# Autodesk Inventor assembly: servoMount
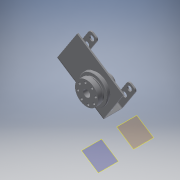
[picture p0: Inventor's stored thumbnail of the model, 180x180]
Saved by Autodesk Inventor 2017 (Build 210142000, 142)
## iProperties
Created: 2017-03-22
Part Number: servoMount
Document SubType Name: Assembly
Designer: admin
Author: admin
## Documents named in this file (5)
- C:\Users\admin\Desktop\CAD\servoMount.iam
- C:\Users\admin\Downloads\bearing.ipt
- C:\Users\admin\Downloads\hub.ipt
- C:\Users\admin\Downloads\Hitec HS-325HB.ipt
- C:\Users\admin\Desktop\CAD\HSmount.ipt
## Components (4 placed, 4 different names)
1. bearing:1 — Mate:3
2. hub:1 — Insert:1, Mate:3
3. Hitec HS-325HB:1 — Insert:1, Mate:1, Mate:2
4. HSmount:1 — Mate:1, Mate:2
## Relationships (4: Mate 3, Insert 1)
- Insert:1: hub:1 ↔ Hitec HS-325HB:1
- Mate:1: Hitec HS-325HB:1 ↔ HSmount:1
- Mate:2: Hitec HS-325HB:1 ↔ HSmount:1
- Mate:3: bearing:1 ↔ hub:1
